# Autodesk Inventor assembly: Top_Arm_Assembly
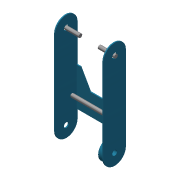
[picture p0: Inventor's stored thumbnail of the model, 180x180]
Saved by Autodesk Inventor 2016 (Build 200138000, 138)
## iProperties
Created: 2015-05-19
Part Number: Top_Arm_Assembly
Document SubType Name: Assembly
Designer: CHUNGBK
Author: CHUNGBK
## Documents named in this file (4)
- C:\Users\jonathan\Desktop\Five Axis Serial Robotic Arm\Inventor\Scorbot Elbow.iam
- C:\Users\jonathan\Desktop\Five Axis Serial Robotic Arm\Inventor\Elbow.ipt
- C:\Users\jonathan\Desktop\Five Axis Serial Robotic Arm\Inventor\Elbow Rod.ipt
- C:\Users\jonathan\Desktop\Five Axis Serial Robotic Arm\Inventor\Elbow Pivot.ipt
## Components (4 placed, 3 different names)
1. Elbow:1 — Flush:1, Flush:2, Flush:3, Mate:1, Mate:2, Mate:3, Mate:4, Flush:4, Mate:5, Flush:5
2. Elbow Rod:1 — Mate:1, Mate:2, Mate:3
3. Elbow Pivot:1 — Mate:4, Flush:4
4. Elbow Pivot:2 — Mate:5, Flush:5
## Relationships (10: Flush 5, Mate 5)
- Flush:1: Elbow:1
- Flush:2: Elbow:1
- Flush:3: Elbow:1
- Mate:1: Elbow:1 ↔ Elbow Rod:1
- Mate:2 (-44.45 mm): Elbow:1 ↔ Elbow Rod:1
- Mate:3 (61.9125 mm): Elbow:1 ↔ Elbow Rod:1
- Mate:4: Elbow:1 ↔ Elbow Pivot:1
- Flush:4 (-36.7388 mm): Elbow:1 ↔ Elbow Pivot:1
- Mate:5: Elbow:1 ↔ Elbow Pivot:2
- Flush:5 (-36.7388 mm): Elbow:1 ↔ Elbow Pivot:2
